# Autodesk Inventor assembly: PlantExample
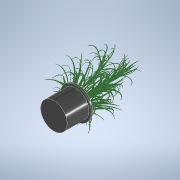
[picture p0: Inventor's stored thumbnail of the model, 180x180]
Saved by Autodesk Inventor 2021 (Build 250183000, 183)
## iProperties
Created: 2021-04-27
Part Number: PlantExample
Document SubType Name: Assembly
Designer: Jorian Brusind
Author: Jorian Brusind
## Documents named in this file (3)
- C:\Users\Jorian Brusind\Documents\GitHub\PersonalProjects\HyperRail\Inventor Files\53083_open3dmodel.com\53083_open3dmodel.com\PlantExample.iam
- C:\Users\Jorian Brusind\Documents\GitHub\PersonalProjects\HyperRail\Inventor Files\53083_open3dmodel.com\53083_open3dmodel.com\7gal.ipt
- C:\Users\Jorian Brusind\Documents\GitHub\PersonalProjects\HyperRail\Inventor Files\53083_open3dmodel.com\53083_open3dmodel.com\Grass N120319.ipt
## Components (2 placed, 2 different names)
1. 7gal:1 — Mate:1, Mate:2, Mate:3
2. Grass N120319:1 — Mate:1
## Relationships (3: Mate 3)
- Mate:1: 7gal:1 ↔ Grass N120319:1
- Mate:2: 7gal:1
- Mate:3: 7gal:1
